# Autodesk Inventor assembly: BaugruppeHalter02
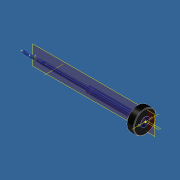
[picture p0: Inventor's stored thumbnail of the model, 180x180]
Saved by Autodesk Inventor 2013 (Build 170138000, 138)
## iProperties
Created: 2006-10-06
Part Number: BaugruppeHalter02
Document SubType Name: Assembly
Designer: acad
Manufacturer: Standard
Standards Organization: Custom
Author: acad
## Documents named in this file (7)
- F:\Halter\Halter_expl.iam
- F:\Halter\Schaft.ipt
- F:\Halter\Kopf.ipt
- F:\Halter\Gabel.ipt
- F:\Halter\Griff.ipt
- F:\Halter\Stift.ipt
- F:\Halter\Blende.ipt
## Components (6 placed, 6 different names)
1. Schaft:1 — Einfügen:1, Einfügen:2, Einfügen:3, Passend:3, Winkel:1, Tangential:2
2. Kopf:1 — Einfügen:2, Passend:1, Tangential:1, Passend:2, Einfügen:4
3. Gabel:1 — Passend:1, Tangential:1, Passend:2, Winkel:1
4. Griff:1 — Einfügen:1, Einfügen:3
5. Stift:1 — Passend:3, Tangential:2
6. Blende:1 — Einfügen:4
## Relationships (10: Insert 4, Mate 3, Tangent 2, Angle 1)
- Einfügen:1 [Insert]: Schaft:1 ↔ Griff:1
- Einfügen:2 [Insert]: Schaft:1 ↔ Kopf:1
- Passend:1 [Mate]: Kopf:1 ↔ Gabel:1
- Tangential:1: Kopf:1 ↔ Gabel:1
- Passend:2 [Mate]: Kopf:1 ↔ Gabel:1
- Einfügen:3 [Insert]: Schaft:1 ↔ Griff:1
- Passend:3 [Mate]: Schaft:1 ↔ Stift:1
- Winkel:1 [Angle] (0 deg): Schaft:1 ↔ Gabel:1
- Einfügen:4 [Insert]: Kopf:1 ↔ Blende:1
- Tangential:2: Schaft:1 ↔ Stift:1
